# Autodesk Inventor assembly: MK4 Swerve Module L1
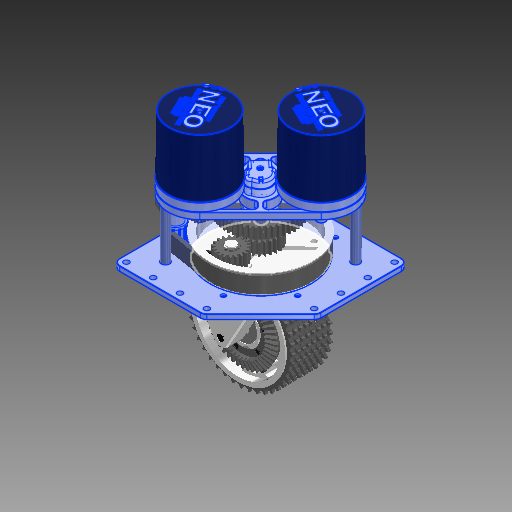
[picture p0: Inventor's stored thumbnail of the model, 512x512]
Saved by Autodesk Inventor 2025 (Build 290162010, 162A)
## iProperties
Created: 2024-07-19
Part Number: MK4 Swerve Module L1
Document SubType Name: Assembly
Designer: rohan
Author: rohan
## Documents named in this file (7)
- D:\ultimate-hecker\Computer-Aided-Design\FRC-Offseason-Design-Training\Parts Library\Drivetrains\Swerve Modules\MK4\MK4 Swerve Module L1.iam
- D:\ultimate-hecker\Computer-Aided-Design\FRC-Offseason-Design-Training\Parts Library\Drivetrains\Swerve Modules\MK4\MK4 Master Structure.iam
- D:\ultimate-hecker\Computer-Aided-Design\FRC-Offseason-Design-Training\Parts Library\Drivetrains\Swerve Modules\MK4\MK4 Turret Assembly L1.iam
- D:\ultimate-hecker\Computer-Aided-Design\FRC-Offseason-Design-Training\Parts Library\Power Transfer\Belts and Pullies\320-5M-15 Belt.ipt
- D:\ultimate-hecker\Computer-Aided-Design\FRC-Offseason-Design-Training\Parts Library\Power Transfer\Gears (Hex)\32T 32DP Spur Gear 375 Hex (SDS).ipt
- D:\ultimate-hecker\Computer-Aided-Design\FRC-Offseason-Design-Training\Parts Library\Power Transfer\Gears (Motor)\SDS-Steel-Spur-Gear (20DP, 8mm Bore, 14T, 14T CD).ipt
- D:\ultimate-hecker\Computer-Aided-Design\FRC-Offseason-Design-Training\Parts Library\Power Transfer\Gears (Motor)\SDS-Steel-Spur-Gear (32DP).ipt
## Components (6 placed, 6 different names)
1. MK4 Master Structure:1 [sub-assembly] — Insert:1, Mate:1, Mate:2, Mate:3, Mate:4, Insert:3, Insert:4, Rotation:2
2. MK4 Turret Assembly L1:1 [sub-assembly] — Insert:1, Insert:2, Rotation:1
3. 320-5M-15 Belt:1 — Insert:2, Mate:1
4. 32T 32DP Spur Gear 375 Hex (SDS):1 — Mate:2, Mate:3, Mate:4
5. SDS-Steel-Spur-Gear (20DP, 8mm Bore, 14T, 14T CD):1 — Insert:3, Rotation:1
6. SDS-Steel-Spur-Gear (32DP):1 — Insert:4, Rotation:2
## Relationships (10: Insert 4, Mate 4, RelateRotation 2)
- Insert:1: MK4 Master Structure:1 ↔ MK4 Turret Assembly L1:1
- Insert:2 (1.651 mm): MK4 Turret Assembly L1:1 ↔ 320-5M-15 Belt:1
- Mate:1: MK4 Master Structure:1 ↔ 320-5M-15 Belt:1
- Mate:2: MK4 Master Structure:1 ↔ 32T 32DP Spur Gear 375 Hex (SDS):1
- Mate:3: MK4 Master Structure:1 ↔ 32T 32DP Spur Gear 375 Hex (SDS):1
- Mate:4: MK4 Master Structure:1 ↔ 32T 32DP Spur Gear 375 Hex (SDS):1
- Insert:3: MK4 Master Structure:1 ↔ SDS-Steel-Spur-Gear (20DP, 8mm Bore, 14T, 14T CD):1
- Rotation:1 [RelateRotation] (0.32 ul): MK4 Turret Assembly L1:1 ↔ SDS-Steel-Spur-Gear (20DP, 8mm Bore, 14T, 14T CD):1
- Insert:4: MK4 Master Structure:1 ↔ SDS-Steel-Spur-Gear (32DP):1
- Rotation:2 [RelateRotation] (0.4688 ul): MK4 Master Structure:1 ↔ SDS-Steel-Spur-Gear (32DP):1
